# Autodesk Inventor assembly: Omniwheel Assembly
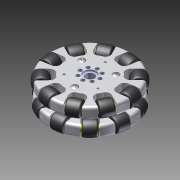
[picture p0: Inventor's stored thumbnail of the model, 180x180]
Saved by Autodesk Inventor 2012 (Build 160160000, 160)
## iProperties
Created: 2011-05-19
Part Number: Omniwheel Assembly
Document SubType Name: Assembly
Designer: Andrew
Author: Andrew
## Documents named in this file (3)
- C:\Users\Andrew\Documents\Inventor\FTC Bots\FTC CAD Database\FTC CAD Files\Wheels\Omniwheel Assembly.iam
- C:\Users\Andrew\Documents\Inventor\FTC Bots\FTC CAD Database\FTC CAD Files\Wheels\3 Inch Omniwheel.iam
- C:\Users\Andrew\Documents\Inventor\FTC Bots\FTC CAD Database\FTC CAD Files\Wheels\Omni Spacer.ipt
## Components (3 placed, 2 different names)
1. 3 Inch Omniwheel:1 [sub-assembly] — Insert:1, Mate:1
2. 3 Inch Omniwheel:2 [sub-assembly] — Mate:2, Mate:3, Mate:4
3. Omni Spacer:1 — Insert:1, Mate:1, Mate:2, Mate:3, Mate:4
## Relationships (5: Mate 4, Insert 1)
- Insert:1: 3 Inch Omniwheel:1 ↔ Omni Spacer:1
- Mate:1: 3 Inch Omniwheel:1 ↔ Omni Spacer:1
- Mate:2: 3 Inch Omniwheel:2 ↔ Omni Spacer:1
- Mate:3: 3 Inch Omniwheel:2 ↔ Omni Spacer:1
- Mate:4: 3 Inch Omniwheel:2 ↔ Omni Spacer:1
